# Autodesk Inventor assembly: Totalen_auto
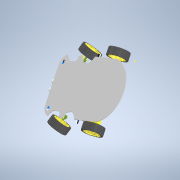
[picture p0: Inventor's stored thumbnail of the model, 180x180]
Saved by Autodesk Inventor 2022 (Build 260153000, 153)
## iProperties
Created: 2021-11-25
Part Number: Totalen_auto
Document SubType Name: Assembly
Designer: keemi
Author: keemi
## Documents named in this file (12)
- C:\Users\keemi\OneDrive\Documents\Inventor\Auto\Totalen_auto.iam
- C:\Users\keemi\OneDrive\Documents\Inventor\Auto\Onderplaat-v1.ipt
- C:\Users\keemi\OneDrive\Documents\Inventor\Auto\esp-32s-electrical-1.snapshot.1\EPS Wroom 3.2 ESP-32S.ipt
- C:\Users\keemi\OneDrive\Documents\Inventor\Auto\geared-dc-motor-for-arduino-applications-1.snapshot.2\Hobi - Motor DC 1.ipt
- C:\Users\keemi\OneDrive\Documents\Inventor\Auto\half-breadboard-1.snapshot.3\HalfBreadboard.ipt
- C:\Users\keemi\OneDrive\Documents\Inventor\Auto\ultrasonic-sensor-hc-sr04-4.snapshot.11\Ultrasonic Sensor HC-SR04\Ultrasonic Sensor HC-SR04.ipt
- C:\Users\keemi\OneDrive\Documents\Inventor\Auto\wheel-arduino-1.snapshot.2\Wheel ALL.ipt
- C:\Users\keemi\OneDrive\Documents\Inventor\Auto\staafje.ipt
- C:\Users\keemi\OneDrive\Documents\Inventor\Auto\stuur_ARMPJE.ipt
- C:\Users\keemi\OneDrive\Documents\Inventor\Auto\ir_sensor-1.snapshot.1\IR sensor.ipt
- C:\Users\keemi\OneDrive\Documents\Inventor\Auto\HENK.ipt
- C:\Users\keemi\OneDrive\Documents\Inventor\Auto\POWERBANK.ipt
## Components (23 placed, 11 different names)
1. Onderplaat-v1:1 — Mate:1, Flush:1, Mate:2, Flush:3, Flush:4, Mate:8, Mate:11, Mate:12, Rigid:1, Rotational:1, Mate:16, Mate:19, Mate:25, Mate:26, Mate:27, Mate:28, Flush:6, Flush:7, Mate:29, Flush:8, Flush:9, Flush:10, Flush:11, Mate:30, Flush:13, Flush:14, Mate:35, Flush:18, Mate:36, Mate:38, Flush:20
2. EPS Wroom 3.2 ESP-32S:1 — Mate:9, Mate:10, Flush:5
3. Hobi - Motor DC 1:1 — Mate:1, Flush:1, Flush:2, Flush:4, Mate:4, Mate:5
4. Hobi - Motor DC 1:2 — Mate:2, Flush:2, Flush:3, Mate:6, Mate:7
5. HalfBreadboard:1 — Mate:8, Mate:9, Mate:10, Flush:5, Flush:18, Mate:37, Flush:19, Flush:20, Flush:21
6. Ultrasonic Sensor HC-SR04:1 — Mate:30, Flush:13, Flush:14
7. Wheel ALL:1 — Mate:4, Mate:5
8. Wheel ALL:2 — Mate:6, Mate:7
9. staafje:1 — Mate:11, Rigid:1, Mate:17
10. staafje:2 — Mate:12, Rotational:1, Mate:24
11. stuur_ARMPJE:1 — Mate:16, Mate:17, Mate:21, Mate:22, Mate:32, Flush:16, Flush:17
12. stuur_ARMPJE:2 — Mate:15, Mate:19, Mate:23, Mate:24, Mate:31, Flush:15
13. Wheel ALL:3 — Mate:21, Mate:22
14. Wheel ALL:4 — Mate:15, Mate:23
15. IR sensor:1 — Mate:28, Flush:8, Flush:9
16. IR sensor:2 — Mate:27, Flush:10, Flush:11
17. IR sensor:3 — Mate:26, Flush:7, Mate:35
18. IR sensor:4 — Mate:25, Flush:6, Mate:29
19. staafje:3 — Mate:32, Mate:33, Flush:16
20. staafje:4 — Mate:31, Mate:34, Flush:15
21. HENK:1 — Mate:33, Mate:34, Flush:17
22. HalfBreadboard:2 — Mate:38, Mate:39, Flush:19
23. POWERBANK:1 — Mate:36, Mate:37, Mate:39, Flush:21
## Relationships (56: Mate 34, Flush 20, WeldJoint 1, RevoluteJoint 1)
- Mate:1: Onderplaat-v1:1 ↔ Hobi - Motor DC 1:1
- Flush:1: Onderplaat-v1:1 ↔ Hobi - Motor DC 1:1
- Mate:2: Onderplaat-v1:1 ↔ Hobi - Motor DC 1:2
- Flush:2: Hobi - Motor DC 1:1 ↔ Hobi - Motor DC 1:2
- Flush:3: Onderplaat-v1:1 ↔ Hobi - Motor DC 1:2
- Flush:4 (210 mm): Onderplaat-v1:1 ↔ Hobi - Motor DC 1:1
- Mate:4: Hobi - Motor DC 1:1 ↔ Wheel ALL:1
- Mate:5 (1 mm): Hobi - Motor DC 1:1 ↔ Wheel ALL:1
- Mate:6 (1 mm): Hobi - Motor DC 1:2 ↔ Wheel ALL:2
- Mate:7: Hobi - Motor DC 1:2 ↔ Wheel ALL:2
- Mate:8: Onderplaat-v1:1 ↔ HalfBreadboard:1
- Mate:9 (1 mm): EPS Wroom 3.2 ESP-32S:1 ↔ HalfBreadboard:1
- Mate:10 (-54 mm): EPS Wroom 3.2 ESP-32S:1 ↔ HalfBreadboard:1
- Flush:5 (13 mm): EPS Wroom 3.2 ESP-32S:1 ↔ HalfBreadboard:1
- Mate:11: Onderplaat-v1:1 ↔ staafje:1
- Mate:12: Onderplaat-v1:1 ↔ staafje:2
- Rigid:1 [WeldJoint]: Onderplaat-v1:1 ↔ staafje:1
- Rotational:1 [RevoluteJoint]: Onderplaat-v1:1 ↔ staafje:2
- Mate:15: stuur_ARMPJE:2 ↔ Wheel ALL:4
- Mate:16 (9 mm): Onderplaat-v1:1 ↔ stuur_ARMPJE:1
- Mate:17: staafje:1 ↔ stuur_ARMPJE:1
- Mate:19 (9 mm): Onderplaat-v1:1 ↔ stuur_ARMPJE:2
- Mate:21 (7 mm): stuur_ARMPJE:1 ↔ Wheel ALL:3
- Mate:22: stuur_ARMPJE:1 ↔ Wheel ALL:3
- Mate:23 (7 mm): stuur_ARMPJE:2 ↔ Wheel ALL:4
- Mate:24: staafje:2 ↔ stuur_ARMPJE:2
- Mate:25: Onderplaat-v1:1 ↔ IR sensor:4
- Mate:26: Onderplaat-v1:1 ↔ IR sensor:3
- Mate:27: Onderplaat-v1:1 ↔ IR sensor:2
- Mate:28: Onderplaat-v1:1 ↔ IR sensor:1
- Flush:6 (8 mm): Onderplaat-v1:1 ↔ IR sensor:4
- Flush:7 (8 mm): Onderplaat-v1:1 ↔ IR sensor:3
- Mate:29: Onderplaat-v1:1 ↔ IR sensor:4
- Flush:8: Onderplaat-v1:1 ↔ IR sensor:1
- Flush:9 (-5 mm): Onderplaat-v1:1 ↔ IR sensor:1
- Flush:10: Onderplaat-v1:1 ↔ IR sensor:2
- Flush:11 (5 mm): Onderplaat-v1:1 ↔ IR sensor:2
- Mate:30: Onderplaat-v1:1 ↔ Ultrasonic Sensor HC-SR04:1
- Flush:13: Onderplaat-v1:1 ↔ Ultrasonic Sensor HC-SR04:1
- Flush:14 (95 mm): Onderplaat-v1:1 ↔ Ultrasonic Sensor HC-SR04:1
- Mate:31: stuur_ARMPJE:2 ↔ staafje:4
- Mate:32: stuur_ARMPJE:1 ↔ staafje:3
- Mate:33: staafje:3 ↔ HENK:1
- Mate:34: staafje:4 ↔ HENK:1
- Flush:15 (-5 mm): stuur_ARMPJE:2 ↔ staafje:4
- Flush:16 (-5 mm): stuur_ARMPJE:1 ↔ staafje:3
- Flush:17 (2.2 mm): stuur_ARMPJE:1 ↔ HENK:1
- Mate:35: Onderplaat-v1:1 ↔ IR sensor:3
- Flush:18 (90 mm): Onderplaat-v1:1 ↔ HalfBreadboard:1
- Mate:36: Onderplaat-v1:1 ↔ POWERBANK:1
- Mate:37 (10 mm): HalfBreadboard:1 ↔ POWERBANK:1
- Mate:38: Onderplaat-v1:1 ↔ HalfBreadboard:2
- Mate:39 (10 mm): HalfBreadboard:2 ↔ POWERBANK:1
- Flush:19: HalfBreadboard:1 ↔ HalfBreadboard:2
- Flush:20 (-55 mm): Onderplaat-v1:1 ↔ HalfBreadboard:1
- Flush:21 (4 mm): HalfBreadboard:1 ↔ POWERBANK:1
